# Autodesk Inventor assembly: Unit_SR-W
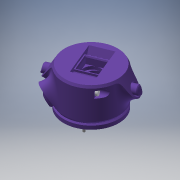
[picture p0: Inventor's stored thumbnail of the model, 180x180]
Saved by Autodesk Inventor 2019.1 (Build 231200000, 200)
## iProperties
Created: 2018-04-24
Part Number: Unit_SR-W
Material: 一般
Document SubType Name: Assembly
Designer: sktom
Author: sktom
## Documents named in this file (13)
- D:\CloudStrage\OneDrive\CADMech\HbSizeSMech\UnitWrist\Unit_SR-W.iam
- D:\CloudStrage\OneDrive\CADMech\HbSizeSMech\UnitWrist\Parts_SR-W\SR-W-04.ipt
- D:\CloudStrage\OneDrive\CADMech\HbSizeSMech\UnitWrist\Parts_SR-W\SR-W-05.ipt
- D:\CloudStrage\OneDrive\CADMech\HbSizeSMech\UnitWrist\Parts_SR-W\SR-W-02.ipt
- D:\CloudStrage\OneDrive\CADMech\HbSizeSMech\UnitWrist\Parts_SR-W\SR-W-08.ipt
- D:\CloudStrage\OneDrive\CADMech\HbSizeSMech\UnitWrist\Parts_SR-W\SR-W-01.ipt
- D:\CloudStrage\OneDrive\CADMech\HbSizeSMech\UnitWrist\Parts_SR-W\SR-W-03.ipt
- D:\CloudStrage\OneDrive\CADMech\HbSizeSMech\UnitWrist\Parts_SR-W\SR-W-06.ipt
- D:\CloudStrage\OneDrive\CADMech\HbSizeSMech\UnitWrist\Parts_SR-W\SR-W-07.ipt
- D:\CloudStrage\OneDrive\CADMech\HbSizeSMech\UnitWrist\Parts_SR-W\Parts_Screw_M2_L6.ipt
- D:\CloudStrage\OneDrive\CADMech\HbSizeSMech\UnitWrist\Parts_SR-W\Parts_Screw_M1.4_L6.ipt
- D:\CloudStrage\OneDrive\CADMech\HbSizeSMech\UnitWrist\Parts_SR-W\Parts_CoilSpring_CP_0.5-4.5-6.5.ipt
- D:\CloudStrage\OneDrive\CADMech\HbSizeSMech\UnitWrist\Parts_SR-W\Parts_Ball_SBM-SUJ-4.5.ipt
## Components (20 placed, 12 different names)
1. SR-W-01:1 — リジッド:1
2. SR-W-02:1 — 挿入:3, 挿入:4, 挿入:5, リジッド:1, 円柱状:1, 挿入:6, 円柱状:2, メイト:1, 挿入:14, 挿入:15, 挿入:16
3. SR-W-03:1 — 円柱状:1, 挿入:6
4. SR-W-04:1 — 挿入:1, 挿入:2, 挿入:3, 挿入:11, 挿入:12, 挿入:13
5. SR-W-05:1 — 挿入:1, 挿入:2, 挿入:9, 挿入:10
6. SR-W-06:1 — リジッド:2
7. SR-W-07:1 — リジッド:2, 円柱状:2, メイト:1
8. SR-W-08:1 — 挿入:4, 挿入:5, 挿入:7, 挿入:8
9. Parts_Screw_M2_L6:1 — 挿入:7
10. Parts_Screw_M2_L6:2 — 挿入:8
11. Parts_Screw_M1.4_L6:1 — 挿入:9
12. Parts_Screw_M1.4_L6:2 — 挿入:10
13. Parts_Screw_M1.4_L6:3 — 挿入:11
14. Parts_Screw_M1.4_L6:4 — 挿入:12
15. Parts_Screw_M1.4_L6:5 — 挿入:13
16. Parts_CoilSpring_CP_0.5-4.5-6.5:1 — 挿入:14
17. Parts_CoilSpring_CP_0.5-4.5-6.5:2 — 挿入:15
18. Parts_CoilSpring_CP_0.5-4.5-6.5:3 — 挿入:16
19. Parts_Ball_SBM-SUJ-4.5:1
20. Parts_Ball_SBM-SUJ-4.5:2
## Relationships (21: Insert 16, WeldJoint 2, CylindricalJoint 2, Mate 1)
- 挿入:1 [Insert]: SR-W-04:1 ↔ SR-W-05:1
- 挿入:2 [Insert]: SR-W-04:1 ↔ SR-W-05:1
- 挿入:3 [Insert]: SR-W-02:1 ↔ SR-W-04:1
- 挿入:4 [Insert]: SR-W-02:1 ↔ SR-W-08:1
- 挿入:5 [Insert]: SR-W-02:1 ↔ SR-W-08:1
- リジッド:1 [WeldJoint]: SR-W-01:1 ↔ SR-W-02:1
- 円柱状:1 [CylindricalJoint]: SR-W-02:1 ↔ SR-W-03:1
- 挿入:6 [Insert]: SR-W-02:1 ↔ SR-W-03:1
- リジッド:2 [WeldJoint]: SR-W-06:1 ↔ SR-W-07:1
- 円柱状:2 [CylindricalJoint]: SR-W-02:1 ↔ SR-W-07:1
- メイト:1 [Mate] (0.5 mm): SR-W-02:1 ↔ SR-W-07:1
- 挿入:7 [Insert]: SR-W-08:1 ↔ Parts_Screw_M2_L6:1
- 挿入:8 [Insert]: SR-W-08:1 ↔ Parts_Screw_M2_L6:2
- 挿入:9 [Insert]: SR-W-05:1 ↔ Parts_Screw_M1.4_L6:1
- 挿入:10 [Insert]: SR-W-05:1 ↔ Parts_Screw_M1.4_L6:2
- 挿入:11 [Insert]: SR-W-04:1 ↔ Parts_Screw_M1.4_L6:3
- 挿入:12 [Insert]: SR-W-04:1 ↔ Parts_Screw_M1.4_L6:4
- 挿入:13 [Insert]: SR-W-04:1 ↔ Parts_Screw_M1.4_L6:5
- 挿入:14 [Insert]: SR-W-02:1 ↔ Parts_CoilSpring_CP_0.5-4.5-6.5:1
- 挿入:15 [Insert]: SR-W-02:1 ↔ Parts_CoilSpring_CP_0.5-4.5-6.5:2
- 挿入:16 [Insert]: SR-W-02:1 ↔ Parts_CoilSpring_CP_0.5-4.5-6.5:3
